# Autodesk Inventor assembly: EL2-.300
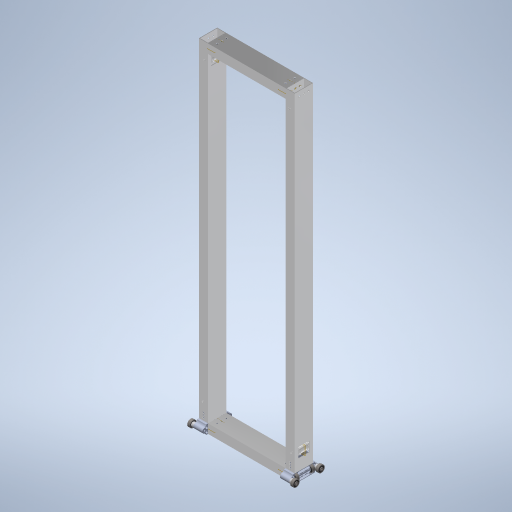
[picture p0: Inventor's stored thumbnail of the model, 512x512]
Saved by Autodesk Inventor 2023.4 (Build 274418000, 418)
## iProperties
Created: 2025-01-11
Part Number: EL2-.300
Document SubType Name: Assembly
Designer: mavericks
Author: mavericks
## Documents named in this file (6)
- C:\Users\mavericks\Documents\Robotics\GitHub\2025-ReefScape---CAD\Elevator\EL2\EL2-.300.iam
- C:\Users\mavericks\Documents\Robotics\GitHub\2025-ReefScape---CAD\Elevator\EL2\EL2-004.ipt
- C:\Users\mavericks\Documents\Robotics\GitHub\2025-ReefScape---CAD\COMMON PARTS\WCP Elevator parts\WCP-0199\WCP-0199.iam
- C:\Users\mavericks\Documents\Robotics\GitHub\2025-ReefScape---CAD\Elevator\EL2\EL2-006.ipt
- C:\Users\mavericks\Documents\Robotics\GitHub\2025-ReefScape---CAD\Elevator\EL2\EL2-005.ipt
- C:\Users\mavericks\Documents\Robotics\GitHub\2025-ReefScape---CAD\Elevator\EL2\EL2-400.iam
## Components (14 placed, 5 different names)
1. EL2-004:1 — Flush:1, Flush:2, Mate:1, Insert:3, Flush:12, Symmetry:1, Insert:4, Insert:6
2. WCP-0199:1 [sub-assembly] — Flush:1, Flush:2, Mate:1, Mate:5, Insert:1
3. EL2-006:1 — Flush:3, Flush:4, Mate:2, Mate:3, Mate:4, Flush:5, Flush:8
4. EL2-005:1 — Flush:3, Flush:4, Mate:2, Mate:5, Insert:2
5. EL2-005:2 — Mate:3, Mate:4, Flush:5, Insert:1
6. EL2-004:2 — Symmetry:1, Insert:5, Insert:7
7. WCP-0199:2 [sub-assembly] — Insert:2, Flush:8
8. EL2-006:3 — Flush:12
9. EL2-005:3
10. EL2-005:4 — Insert:3
11. EL2-400:1 [sub-assembly] — Insert:5
12. EL2-400:2 [sub-assembly] — Insert:4
13. EL2-400:3 [sub-assembly] — Insert:6
14. EL2-400:4 [sub-assembly] — Insert:7
## Relationships (29: Flush 12, Mate 9, Insert 7, Symmetry 1)
- Flush:1: EL2-004:1 ↔ WCP-0199:1
- Flush:2: EL2-004:1 ↔ WCP-0199:1
- Mate:1: EL2-004:1 ↔ WCP-0199:1
- Flush:3: EL2-006:1 ↔ EL2-005:1
- Flush:4: EL2-006:1 ↔ EL2-005:1
- Mate:2: EL2-006:1 ↔ EL2-005:1
- Mate:3: EL2-006:1 ↔ EL2-005:2
- Mate:4: EL2-006:1 ↔ EL2-005:2
- Flush:5: EL2-006:1 ↔ EL2-005:2
- Mate:5: WCP-0199:1 ↔ EL2-005:1
- Insert:1: WCP-0199:1 ↔ EL2-005:2
- [Flush]: EL2-004:2 ↔ WCP-0199:2
- [Flush]: EL2-004:2 ↔ WCP-0199:2
- [Mate]: EL2-004:2 ↔ WCP-0199:2
- Insert:2: EL2-005:1 ↔ WCP-0199:2
- Flush:8: EL2-006:1 ↔ WCP-0199:2
- [Flush]: EL2-006:3 ↔ EL2-005:3
- [Flush]: EL2-006:3 ↔ EL2-005:3
- [Mate]: EL2-006:3 ↔ EL2-005:3
- [Mate]: EL2-006:3 ↔ EL2-005:4
- [Mate]: EL2-006:3 ↔ EL2-005:4
- [Flush]: EL2-006:3 ↔ EL2-005:4
- Insert:3: EL2-004:1 ↔ EL2-005:4
- Flush:12: EL2-004:1 ↔ EL2-006:3
- Symmetry:1: EL2-004:1 ↔ EL2-004:2
- Insert:4: EL2-004:1 ↔ EL2-400:2
- Insert:5: EL2-004:2 ↔ EL2-400:1
- Insert:6: EL2-004:1 ↔ EL2-400:3
- Insert:7: EL2-004:2 ↔ EL2-400:4
## Named parameters: d11_d0 = 0 mm, d12_d1 = 0 mm, d13_d2 = 0 mm, d16_d3 = 0 mm, d17_d4 = 0 mm, d18_d5 = 0 mm, d19_d6 = 0 mm, d20_d7 = 0 mm, d21_d8 = 0 mm
